# Autodesk Inventor assembly: Robot Chassis 2014
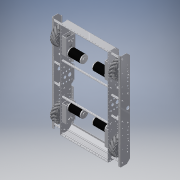
[picture p0: Inventor's stored thumbnail of the model, 180x180]
Saved by Autodesk Inventor 2016 (Build 200138000, 138)
## iProperties
Created: 2014-01-08
Part Number: Robot Chassis 2014
Document SubType Name: Assembly
Designer: 300593
Mass: 2050.24 g
Surface Area: 25894.1 cm^2
Volume: 4905.32 cm^3
Translation Standard: STEP AP203
FileName: AM14U Long and AM14U Wide.STEP
PreProcessor: SolidWorks 2010
PostProcessor: Build: 138, Release: 2013 RTM - Date: Thu 03/01/2012
Sent Units: inch
Uncertainty: 1e-05
Author: 300593
## Documents named in this file (5)
- \\Mac\Home\Desktop\bunnybots 2016\15102898-16-Bunnybot-CAD\Bunnybot-To_be_renamed\15102898-16-A-0000\15102898-16-A-0100\15102898-16-A-0100.iam
- \\Mac\Home\Desktop\bunnybots 2016\15102898-16-Bunnybot-CAD\Bunnybot-To_be_renamed\15102898-16-A-0000\15102898-16-A-0100\AM14U Long.iam
- \\Mac\Home\Desktop\bunnybots 2016\15102898-16-Bunnybot-CAD\Bunnybot-To_be_renamed\15102898-16-A-0000\15102898-16-A-0100\Left-6-inch-HD-Mecanum-Wheel.iam
- \\Mac\Home\Desktop\bunnybots 2016\15102898-16-Bunnybot-CAD\Bunnybot-To_be_renamed\15102898-16-A-0000\15102898-16-A-0100\Right-6-inch-HD-Mecanum-Wheel.iam
- \\Mac\Home\Desktop\bunnybots 2016\15102898-16-Bunnybot-CAD\Bunnybot-To_be_renamed\15102898-16-A-0000\15102898-16-A-0100\Toughbox-nano-hex-asm.iam
## Components (9 placed, 4 different names)
1. AM14U Long:1 [sub-assembly] — Mate:1, Mate:2, Mate:3, Mate:4, Mate:5, Mate:6, Mate:7, Mate:8, Mate:9, Mate:10, Mate:11, Mate:12, Mate:17, Mate:18, Mate:19, Mate:20
2. Left-6-inch-HD-Mecanum-Wheel:1 [sub-assembly] — Mate:16, Mate:17
3. Left-6-inch-HD-Mecanum-Wheel:2 [sub-assembly] — Mate:14, Mate:20
4. Right-6-inch-HD-Mecanum-Wheel:1 [sub-assembly] — Mate:13, Mate:19
5. Right-6-inch-HD-Mecanum-Wheel:2 [sub-assembly] — Mate:15, Mate:18
6. Toughbox-nano-hex-asm:1 [sub-assembly] — Mate:7, Mate:10, Mate:12, Mate:13
7. Toughbox-nano-hex-asm:2 [sub-assembly] — Mate:8, Mate:9, Mate:11, Mate:14
8. Toughbox-nano-hex-asm:3 [sub-assembly] — Mate:4, Mate:5, Mate:6, Mate:15
9. Toughbox-nano-hex-asm:4 [sub-assembly] — Mate:1, Mate:2, Mate:3, Mate:16
## Relationships (20: Mate 20)
- Mate:1: AM14U Long:1 ↔ Toughbox-nano-hex-asm:4
- Mate:2: AM14U Long:1 ↔ Toughbox-nano-hex-asm:4
- Mate:3: AM14U Long:1 ↔ Toughbox-nano-hex-asm:4
- Mate:4: AM14U Long:1 ↔ Toughbox-nano-hex-asm:3
- Mate:5: AM14U Long:1 ↔ Toughbox-nano-hex-asm:3
- Mate:6: AM14U Long:1 ↔ Toughbox-nano-hex-asm:3
- Mate:7: AM14U Long:1 ↔ Toughbox-nano-hex-asm:1
- Mate:8: AM14U Long:1 ↔ Toughbox-nano-hex-asm:2
- Mate:9: AM14U Long:1 ↔ Toughbox-nano-hex-asm:2
- Mate:10: AM14U Long:1 ↔ Toughbox-nano-hex-asm:1
- Mate:11: AM14U Long:1 ↔ Toughbox-nano-hex-asm:2
- Mate:12: AM14U Long:1 ↔ Toughbox-nano-hex-asm:1
- Mate:13: Right-6-inch-HD-Mecanum-Wheel:1 ↔ Toughbox-nano-hex-asm:1
- Mate:14: Left-6-inch-HD-Mecanum-Wheel:2 ↔ Toughbox-nano-hex-asm:2
- Mate:15: Right-6-inch-HD-Mecanum-Wheel:2 ↔ Toughbox-nano-hex-asm:3
- Mate:16: Left-6-inch-HD-Mecanum-Wheel:1 ↔ Toughbox-nano-hex-asm:4
- Mate:17 (19.3294 mm): AM14U Long:1 ↔ Left-6-inch-HD-Mecanum-Wheel:1
- Mate:18 (19.3294 mm): AM14U Long:1 ↔ Right-6-inch-HD-Mecanum-Wheel:2
- Mate:19 (19.3294 mm): AM14U Long:1 ↔ Right-6-inch-HD-Mecanum-Wheel:1
- Mate:20 (19.3294 mm): AM14U Long:1 ↔ Left-6-inch-HD-Mecanum-Wheel:2
